# Autodesk Inventor assembly: kinect_ring
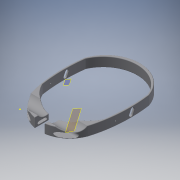
[picture p0: Inventor's stored thumbnail of the model, 180x180]
Saved by Autodesk Inventor 2019 (Build 230136000, 136)
## iProperties
Created: 2024-05-02
Part Number: kinect_ring
Material: Generisch
Document SubType Name: Assembly
Designer: nic
Author: nic
## Documents named in this file (2)
- C:\Users\Nicolas Frick\Sync\OneDrive\wtm\nias\nias_description\inventor_files\kinect_ring.iam
- C:\Users\Nicolas Frick\Sync\OneDrive\wtm\nias\nias_description\inventor_files\kinect_ring.ipt
## Components (1 placed, 1 different names)
1. kinect_ring:1 — Passend:1
## Relationships (1: Mate 1)
- Passend:1 [Mate]: kinect_ring:1
